# Autodesk Inventor assembly: Механизм№2 (разраб)
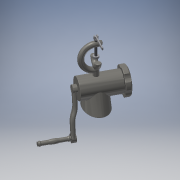
[picture p0: Inventor's stored thumbnail of the model, 180x180]
Saved by Autodesk Inventor 2019 (Build 230136000, 136)
## iProperties
Created: 2019-04-27
Part Number: Механизм№2 (разраб)
Material: Типовые
Document SubType Name: Assembly
Designer: BarmanKaktus
Author: BarmanKaktus
## Documents named in this file (10)
- E:\Автодоска\файлы из доски\мясорубка\Механизм№2 (разраб).iam
- E:\Автодоска\файлы из доски\мясорубка\Корпус.ipt
- E:\Автодоска\файлы из доски\мясорубка\Шнек.ipt
- E:\Автодоска\файлы из доски\мясорубка\Нож.ipt
- E:\Автодоска\файлы из доски\мясорубка\Матрица.ipt
- E:\Автодоска\файлы из доски\мясорубка\Крышка М.ipt
- E:\Автодоска\файлы из доски\мясорубка\Рукоядь.ipt
- E:\Автодоска\файлы из доски\мясорубка\Рукаядь рукоядки.ipt
- E:\Автодоска\файлы из доски\мясорубка\опора.ipt
- E:\Автодоска\файлы из доски\мясорубка\зажим.iam
## Components (9 placed, 9 different names)
1. Корпус:1 — Совмещение:1, Совмещение:2, Совмещение:7, Совмещение:8, Угол:13, Заподлицо:7, Совмещение:13, Цилиндрический:1, Цилиндрический:2
2. Шнек:1 — Совмещение:1, Совмещение:2, Угол:9, Заподлицо:3, Заподлицо:4, Заподлицо:5, Совмещение:9, Угол:10, Угол:11, Угол:12, Совмещение:10, Заподлицо:6, Совмещение:11
3. Нож:1 — Угол:11, Угол:12, Совмещение:10, Заподлицо:6
4. Матрица:1 — Угол:13, Заподлицо:7, Совмещение:11
5. Крышка М:1 — Совмещение:7, Совмещение:8
6. Рукоядь:1 — Угол:9, Заподлицо:3, Заподлицо:4, Заподлицо:5, Совмещение:9, Угол:10, Угол:14, Заподлицо:8, Совмещение:12
7. Рукаядь рукоядки:1 — Угол:14, Заподлицо:8, Совмещение:12
8. зажим:1 [sub-assembly] — Совмещение:13, Угол:15, Совмещение:14, Совмещение:15, Цилиндрический:2
9. опора:1 — Угол:15, Совмещение:14, Совмещение:15, Цилиндрический:1
## Relationships (26: Mate 11, Angle 7, Flush 6, CylindricalJoint 2)
- Совмещение:1 [Mate]: Корпус:1 ↔ Шнек:1
- Совмещение:2 [Mate]: Корпус:1 ↔ Шнек:1
- Совмещение:7 [Mate]: Корпус:1 ↔ Крышка М:1
- Совмещение:8 [Mate]: Корпус:1 ↔ Крышка М:1
- Угол:9 [Angle] (130.63 deg): Шнек:1 ↔ Рукоядь:1
- Заподлицо:3 [Flush]: Шнек:1 ↔ Рукоядь:1
- Заподлицо:4 [Flush]: Шнек:1 ↔ Рукоядь:1
- Заподлицо:5 [Flush]: Шнек:1 ↔ Рукоядь:1
- Совмещение:9 [Mate]: Шнек:1 ↔ Рукоядь:1
- Угол:10 [Angle] (180 deg): Шнек:1 ↔ Рукоядь:1
- Угол:11 [Angle] (0 deg): Шнек:1 ↔ Нож:1
- Угол:12 [Angle] (0 deg): Шнек:1 ↔ Нож:1
- Совмещение:10 [Mate]: Шнек:1 ↔ Нож:1
- Заподлицо:6 [Flush]: Шнек:1 ↔ Нож:1
- Угол:13 [Angle] (180 deg): Корпус:1 ↔ Матрица:1
- Заподлицо:7 [Flush] (-2 mm): Корпус:1 ↔ Матрица:1
- Совмещение:11 [Mate]: Шнек:1 ↔ Матрица:1
- Угол:14 [Angle] (180 deg): Рукоядь:1 ↔ Рукаядь рукоядки:1
- Заподлицо:8 [Flush]: Рукоядь:1 ↔ Рукаядь рукоядки:1
- Совмещение:12 [Mate]: Рукоядь:1 ↔ Рукаядь рукоядки:1
- Совмещение:13 [Mate]: Корпус:1 ↔ зажим:1
- Угол:15 [Angle] (180 deg): зажим:1 ↔ опора:1
- Совмещение:14 [Mate]: зажим:1 ↔ опора:1
- Совмещение:15 [Mate]: зажим:1 ↔ опора:1
- Цилиндрический:1 [CylindricalJoint]: Корпус:1 ↔ опора:1
- Цилиндрический:2 [CylindricalJoint]: Корпус:1 ↔ зажим:1
